# Autodesk Inventor assembly: kiteAssembly
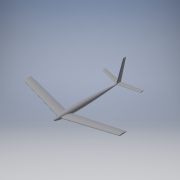
[picture p0: Inventor's stored thumbnail of the model, 180x180]
Saved by Autodesk Inventor 2019.3 (Build 233278000, 278)
## iProperties
Created: 2019-06-24
Part Number: kiteAssembly
Document SubType Name: Assembly
Designer: asiddiq2
Mass: 1.88995e+06 g
Surface Area: 324966 cm^2
Volume: 1.88995e+06 cm^3
Density: 1 g/cm^3
Author: asiddiq2
## Documents named in this file (5)
- C:\Users\asiddiq2\Desktop\OCT_project\CAD_models\kite\kiteAssembly.iam
- C:\Users\asiddiq2\Desktop\OCT_project\CAD_models\kite\camberedWing.ipt
- C:\Users\asiddiq2\Desktop\OCT_project\CAD_models\kite\symmetricHS.ipt
- C:\Users\asiddiq2\Desktop\OCT_project\CAD_models\kite\symmetricVS.ipt
- C:\Users\asiddiq2\Desktop\OCT_project\CAD_models\kite\fuselage.ipt
## Components (4 placed, 4 different names)
1. camberedWing:1 — Flush:1, Flush:2, Flush:5, Flush:6, Flush:7, Flush:8
2. symmetricHS:1 — Flush:1, Flush:2, Flush:3, Mate:1, Flush:4, Flush:5, Flush:9
3. symmetricVS:1 — Flush:3, Mate:1, Flush:4
4. fuselage:1 — Mate:2, Mate:3, Flush:9
## Relationships (12: Flush 9, Mate 3)
- Flush:1: camberedWing:1 ↔ symmetricHS:1
- Flush:2: camberedWing:1 ↔ symmetricHS:1
- Flush:3: symmetricHS:1 ↔ symmetricVS:1
- Mate:1: symmetricHS:1 ↔ symmetricVS:1
- Flush:4: symmetricHS:1 ↔ symmetricVS:1
- Flush:5 (6000 mm): camberedWing:1 ↔ symmetricHS:1
- Flush:6: camberedWing:1
- Flush:7: camberedWing:1
- Flush:8: camberedWing:1
- Mate:2: fuselage:1
- Mate:3: fuselage:1
- Flush:9: symmetricHS:1 ↔ fuselage:1
